# Autodesk Inventor assembly: Rear B
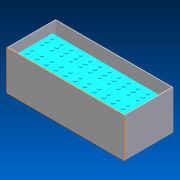
[picture p0: Inventor's stored thumbnail of the model, 180x180]
Saved by Autodesk Inventor 2012 (Build 160160000, 160)
## iProperties
Created: 2012-07-01
Part Number: Rear B
Document SubType Name: Assembly
Designer: Hemant
Author: Hemant
## Documents named in this file (3)
- C:\Users\Hemant\Documents\Bat Boxes COmplete\Rear B.iam
- C:\Users\Hemant\Documents\super large Battery Box Pastic 4.ipt
- C:\Users\Hemant\Documents\CALB100AH.ipt
## Components (25 placed, 2 different names)
1. super large Battery Box Pastic 4:1 — Mate:1, Mate:2, Mate:3
2. CALB100AH:1
3. CALB100AH:2 — Mate:2
4. CALB100AH:3
5. CALB100AH:4
6. CALB100AH:5
7. CALB100AH:6
8. CALB100AH:7
9. CALB100AH:8
10. CALB100AH:9
11. CALB100AH:10 — Mate:3
12. CALB100AH:11
13. CALB100AH:12
14. CALB100AH:13
15. CALB100AH:14
16. CALB100AH:15
17. CALB100AH:16
18. CALB100AH:17
19. CALB100AH:18
20. CALB100AH:19
21. CALB100AH:20 — Mate:1
22. CALB100AH:21
23. CALB100AH:22
24. CALB100AH:23
25. CALB100AH:24
## Component patterns: (12 elements), (2 elements, first: CALB100AH:1), Component Pattern 1:2 (2 elements), Component Pattern 1:3 (2 elements), Component Pattern 1:4 (2 elements), Component Pattern 1:5 (2 elements), Component Pattern 1:6 (2 elements), Component Pattern 1:7 (2 elements), Component Pattern 1:8 (2 elements), Component Pattern 1:9 (2 elements), Component Pattern 1:10 (2 elements), Component Pattern 1:11 (2 elements), Component Pattern 1:12 (2 elements)
## Relationships (3: Mate 3)
- Mate:1: super large Battery Box Pastic 4:1 ↔ CALB100AH:20
- Mate:2 (5.1435 mm): super large Battery Box Pastic 4:1 ↔ CALB100AH:2
- Mate:3 (27.4955 mm): super large Battery Box Pastic 4:1 ↔ CALB100AH:10
